# Autodesk Inventor assembly: GFRP_T2_18
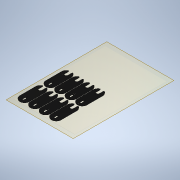
[picture p0: Inventor's stored thumbnail of the model, 180x180]
Saved by Autodesk Inventor 2020 (Build 240168000, 168)
## iProperties
Created: 2021-08-27
Part Number: GFRP_T2_18
Document SubType Name: Assembly
Designer: Masato
Author: Masato
## Documents named in this file (3)
- D:\GitHub\inventor\SUSTAINA-OP\Cam\GFRP_T2_18.iam
- D:\GitHub\inventor\SUSTAINA-OP\Cam\DisposableBoard.ipt
- D:\GitHub\inventor\SUSTAINA-OP\UpperBody\Arm\ForeArm_inside_frame.ipt
## Components (9 placed, 2 different names)
1. DisposableBoard:1 — メイト:2, メイト:1, フラッシュ:1, フラッシュ:2, メイト:4, 正接:1, メイト:5
2. ForeArm_inside_frame:1 — メイト:4, 正接:1, メイト:5
3. ForeArm_inside_frame:2
4. ForeArm_inside_frame:3
5. ForeArm_inside_frame:4
6. ForeArm_inside_frame:5
7. ForeArm_inside_frame:6
8. ForeArm_inside_frame:7
9. ForeArm_inside_frame:8
## Component patterns: (8 elements, first: ForeArm_inside_frame:1)
## Relationships (7: Mate 4, Flush 2, Tangent 1)
- メイト:2 [Mate]: DisposableBoard:1
- メイト:1 [Mate]: DisposableBoard:1
- フラッシュ:1 [Flush]: DisposableBoard:1
- フラッシュ:2 [Flush]: DisposableBoard:1
- メイト:4 [Mate]: DisposableBoard:1 ↔ ForeArm_inside_frame:1
- 正接:1 [Tangent] (2 mm): DisposableBoard:1 ↔ ForeArm_inside_frame:1
- メイト:5 [Mate] (2 mm): DisposableBoard:1 ↔ ForeArm_inside_frame:1
